# Autodesk Inventor assembly: Shoulder
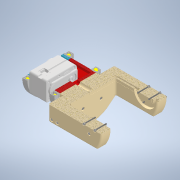
[picture p0: Inventor's stored thumbnail of the model, 180x180]
Saved by Autodesk Inventor 2021 (Build 250183000, 183)
## iProperties
Created: 2020-02-11
Part Number: Shoulder
Document SubType Name: Assembly
Designer: JochenAlt
Author: JochenAlt
## Documents named in this file (6)
- C:\Users\Jochen Alt\Documents\Daten\Projects\MiniBot\CAD\Shoulder.iam
- C:\Users\Jochen Alt\Documents\Daten\Projects\MiniBot\CAD\extern\bearings\65x85x10\61813-2RS1.iam
- C:\Users\Jochen Alt\Documents\Daten\Projects\MiniBot\CAD\extern\Herkulex\Herkulex DRS-040x.ipt
- C:\Users\Jochen Alt\Documents\Daten\Projects\MiniBot\CAD\Shoulder.ipt
- D:\Projects\MiniBot\CAD\extern\DIN 912\DIN 912 - M2 x 0,4 x 20 x 19.ipt
- D:\Projects\MiniBot\CAD\extern\DIN 912\DIN 912 - M2 x 0.4 x 10 x 9.ipt
## Components (28 placed, 5 different names)
1. 61813-2RS1:1 [sub-assembly] — Passend:7, Passend:10
2. 61813-2RS1:2 [sub-assembly] — Passend:8, Passend:11
3. Herkulex DRS-040x:1 — Passend:9, Passend:13, Winkel:1
4. Shoulder:1 — Passend:7, Passend:8, Passend:9, Passend:10, Passend:11, Passend:13, Winkel:1, Insert:1, Insert:2, Insert:3, Insert:4, Insert:5, Insert:6, Insert:7, Insert:8, Insert:9, Insert:10, Insert:11, Insert:12, Insert:13, Insert:14, Insert:15, Insert:16, Insert:17, Insert:18, Insert:19, Insert:20, Insert:21, Insert:26, Insert:27, Insert:28
5. DIN 912 - replaced by DIN EN ISO 4762 M2 x 20:1 — Insert:1
6. DIN 912 - replaced by DIN EN ISO 4762 M2 x 20:2 — Insert:2
7. DIN 912 - replaced by DIN EN ISO 4762 M2 x 20:3 — Insert:3
8. DIN 912 - replaced by DIN EN ISO 4762 M2 x 20:4 — Insert:4
9. DIN 912 - replaced by DIN EN ISO 4762 M2 x 10:1 — Insert:5
10. DIN 912 - replaced by DIN EN ISO 4762 M2 x 10:2 — Insert:6
11. DIN 912 - replaced by DIN EN ISO 4762 M2 x 10:3 — Insert:7
12. DIN 912 - replaced by DIN EN ISO 4762 M2 x 10:4 — Insert:8
13. DIN 912 - replaced by DIN EN ISO 4762 M2 x 10:5 — Insert:9
14. DIN 912 - replaced by DIN EN ISO 4762 M2 x 10:6 — Insert:10
15. DIN 912 - replaced by DIN EN ISO 4762 M2 x 10:7 — Insert:11
16. DIN 912 - replaced by DIN EN ISO 4762 M2 x 10:8 — Insert:12
17. DIN 912 - replaced by DIN EN ISO 4762 M2 x 20:5 — Insert:13
18. DIN 912 - replaced by DIN EN ISO 4762 M2 x 20:6 — Insert:14
19. DIN 912 - replaced by DIN EN ISO 4762 M2 x 20:7 — Insert:15
20. DIN 912 - replaced by DIN EN ISO 4762 M2 x 20:8 — Insert:16
21. DIN 912 - replaced by DIN EN ISO 4762 M2 x 20:9 — Insert:17
22. DIN 912 - replaced by DIN EN ISO 4762 M2 x 20:10 — Insert:18
23. DIN 912 - replaced by DIN EN ISO 4762 M2 x 20:11 — Insert:19
24. DIN 912 - replaced by DIN EN ISO 4762 M2 x 20:12 — Insert:20
25. DIN 912 - replaced by DIN EN ISO 4762 M2 x 10:9 — Insert:21
26. DIN 912 - replaced by DIN EN ISO 4762 M2 x 10:10 — Insert:26
27. DIN 912 - replaced by DIN EN ISO 4762 M2 x 10:11 — Insert:27
28. DIN 912 - replaced by DIN EN ISO 4762 M2 x 10:12 — Insert:28
## Relationships (31: Insert 24, Mate 6, Angle 1)
- Passend:7 [Mate]: 61813-2RS1:1 ↔ Shoulder:1
- Passend:8 [Mate]: 61813-2RS1:2 ↔ Shoulder:1
- Passend:9 [Mate]: Herkulex DRS-040x:1 ↔ Shoulder:1
- Passend:10 [Mate]: 61813-2RS1:1 ↔ Shoulder:1
- Passend:11 [Mate]: 61813-2RS1:2 ↔ Shoulder:1
- Passend:13 [Mate]: Herkulex DRS-040x:1 ↔ Shoulder:1
- Winkel:1 [Angle] (-90 deg): Herkulex DRS-040x:1 ↔ Shoulder:1
- Insert:1: Shoulder:1 ↔ DIN 912 - replaced by DIN EN ISO 4762 M2 x 20:1
- Insert:2: Shoulder:1 ↔ DIN 912 - replaced by DIN EN ISO 4762 M2 x 20:2
- Insert:3: Shoulder:1 ↔ DIN 912 - replaced by DIN EN ISO 4762 M2 x 20:3
- Insert:4: Shoulder:1 ↔ DIN 912 - replaced by DIN EN ISO 4762 M2 x 20:4
- Insert:5: Shoulder:1 ↔ DIN 912 - replaced by DIN EN ISO 4762 M2 x 10:1
- Insert:6: Shoulder:1 ↔ DIN 912 - replaced by DIN EN ISO 4762 M2 x 10:2
- Insert:7: Shoulder:1 ↔ DIN 912 - replaced by DIN EN ISO 4762 M2 x 10:3
- Insert:8: Shoulder:1 ↔ DIN 912 - replaced by DIN EN ISO 4762 M2 x 10:4
- Insert:9: Shoulder:1 ↔ DIN 912 - replaced by DIN EN ISO 4762 M2 x 10:5
- Insert:10: Shoulder:1 ↔ DIN 912 - replaced by DIN EN ISO 4762 M2 x 10:6
- Insert:11: Shoulder:1 ↔ DIN 912 - replaced by DIN EN ISO 4762 M2 x 10:7
- Insert:12: Shoulder:1 ↔ DIN 912 - replaced by DIN EN ISO 4762 M2 x 10:8
- Insert:13: Shoulder:1 ↔ DIN 912 - replaced by DIN EN ISO 4762 M2 x 20:5
- Insert:14: Shoulder:1 ↔ DIN 912 - replaced by DIN EN ISO 4762 M2 x 20:6
- Insert:15: Shoulder:1 ↔ DIN 912 - replaced by DIN EN ISO 4762 M2 x 20:7
- Insert:16: Shoulder:1 ↔ DIN 912 - replaced by DIN EN ISO 4762 M2 x 20:8
- Insert:17: Shoulder:1 ↔ DIN 912 - replaced by DIN EN ISO 4762 M2 x 20:9
- Insert:18: Shoulder:1 ↔ DIN 912 - replaced by DIN EN ISO 4762 M2 x 20:10
- Insert:19: Shoulder:1 ↔ DIN 912 - replaced by DIN EN ISO 4762 M2 x 20:11
- Insert:20: Shoulder:1 ↔ DIN 912 - replaced by DIN EN ISO 4762 M2 x 20:12
- Insert:21: Shoulder:1 ↔ DIN 912 - replaced by DIN EN ISO 4762 M2 x 10:9
- Insert:26: Shoulder:1 ↔ DIN 912 - replaced by DIN EN ISO 4762 M2 x 10:10
- Insert:27: Shoulder:1 ↔ DIN 912 - replaced by DIN EN ISO 4762 M2 x 10:11
- Insert:28: Shoulder:1 ↔ DIN 912 - replaced by DIN EN ISO 4762 M2 x 10:12
